# Autodesk Inventor assembly: RollerAxleWasherSubAssembly
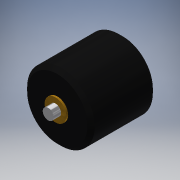
[picture p0: Inventor's stored thumbnail of the model, 180x180]
Saved by Autodesk Inventor 2016 (Build 200138000, 138)
## iProperties
Created: 2016-12-01
Part Number: RollerAxleWasherSubAssembly
Document SubType Name: Assembly
Designer: Evan Phil George
Author: Evan Phil George
## Documents named in this file (4)
- C:\Users\Evan Phil George\Desktop\Ball Balancing Robot\TestBenchInventor\OmniWheel\RollerAxleWasherSubAssembly.iam
- C:\Users\Evan Phil George\Desktop\Ball Balancing Robot\TestBenchInventor\OmniWheel\RollerAxle.ipt
- C:\Users\Evan Phil George\Desktop\Ball Balancing Robot\TestBenchInventor\OmniWheel\Roller.ipt
- C:\Users\Evan Phil George\Desktop\Ball Balancing Robot\TestBenchInventor\OmniWheel\RollerWasher.ipt
## Components (4 placed, 3 different names)
1. RollerAxle:1 — Mate:5, Flush:1
2. Roller:1 — Mate:1, Mate:2, Mate:3, Mate:4, Mate:5, Flush:1
3. RollerWasher:1 — Mate:1, Mate:3
4. RollerWasher:2 — Mate:2, Mate:4
## Relationships (6: Mate 5, Flush 1)
- Mate:1: Roller:1 ↔ RollerWasher:1
- Mate:2: Roller:1 ↔ RollerWasher:2
- Mate:3: Roller:1 ↔ RollerWasher:1
- Mate:4: Roller:1 ↔ RollerWasher:2
- Mate:5: RollerAxle:1 ↔ Roller:1
- Flush:1 (-2.5 mm): RollerAxle:1 ↔ Roller:1
